# Autodesk Inventor assembly: Control Assembly Exploded
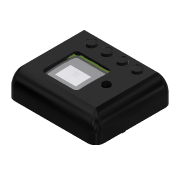
[picture p0: Inventor's stored thumbnail of the model, 180x180]
Saved by Autodesk Inventor 2017 (Build 210142000, 142)
## iProperties
Created: 2016-12-22
Part Number: Control Assembly Exploded
Document SubType Name: Assembly
Designer: ge937963
Author: ge937963
## Documents named in this file (15)
- C:\Users\ge937963\Desktop\Inventor View\Control Assembly.iam
- C:\Users\ge937963\Desktop\Inventor View\Control Board.ipt
- C:\Users\ge937963\Desktop\Inventor View\7 Pin female.iam
- C:\Users\ge937963\Desktop\Inventor View\7 Pin Male.iam
- C:\Users\ge937963\Desktop\Inventor View\Faceplate.ipt
- C:\Users\ge937963\Desktop\Inventor View\Button Piece.ipt
- C:\Users\ge937963\Desktop\Inventor View\Button.ipt
- C:\Users\ge937963\Desktop\Inventor View\2 Pin Female.iam
- C:\Users\ge937963\Desktop\Inventor View\2 Pin Male.iam
- C:\Users\ge937963\Desktop\Inventor View\Power switch.ipt
- C:\Users\ge937963\Desktop\Inventor View\Main PCB.ipt
- C:\Users\ge937963\Desktop\Inventor View\8 Pin female.iam
- C:\Users\ge937963\Desktop\Inventor View\4 Pin Female.iam
- C:\Users\ge937963\Desktop\Inventor View\MicroView.ipt
- C:\Users\ge937963\Desktop\Inventor View\Screw.ipt
## Components (27 placed, 14 different names)
1. Control Board:1 — Mate:52, Mate:53
2. 7 Pin female:1 [sub-assembly] — Mate:48, Mate:49, Mate:51
3. 7 Pin Male:1 [sub-assembly] — Mate:48, Mate:49, Mate:51
4. Faceplate:1 — Mate:53
5. Button Piece:1
6. Button Piece:2
7. Button Piece:3
8. Button Piece:4
9. Button:1
10. Button:2
11. Button:3
12. Button:4
13. 2 Pin Female:1 [sub-assembly]
14. 2 Pin Male:1 [sub-assembly]
15. Power switch:1
16. Main PCB:1
17. 8 Pin female:1 [sub-assembly]
18. 8 Pin female:2 [sub-assembly] — Mate:50
19. 2 Pin Female:2 [sub-assembly]
20. 4 Pin Female:1 [sub-assembly]
21. 4 Pin Female:2 [sub-assembly]
22. 2 Pin Female:3 [sub-assembly]
23. 2 Pin Female:4 [sub-assembly]
24. MicroView:1 — Mate:50
25. Screw:1 — Mate:52
26. Screw:2
27. Screw:3
## Relationships (71: Mate 53, Flush 16, Angle 2)
- [Mate]: Control Board:1 ↔ 7 Pin Male:1
- [Mate]: Control Board:1 ↔ 7 Pin Male:1
- [Mate]: Control Board:1 ↔ Faceplate:1
- [Mate]: Control Board:1 ↔ Faceplate:1
- [Flush]: Button Piece:1 ↔ Button Piece:2
- [Flush]: Button Piece:2 ↔ Button Piece:3
- [Flush]: Button Piece:3 ↔ Button Piece:4
- [Mate]: Faceplate:1 ↔ Button Piece:1
- [Mate]: Faceplate:1 ↔ Button Piece:2
- [Mate]: Faceplate:1 ↔ Button Piece:3
- [Mate]: Faceplate:1 ↔ Button Piece:4
- [Mate]: Control Board:1 ↔ 7 Pin Male:1
- [Flush]: Button:1 ↔ Button:2
- [Flush]: Button:2 ↔ Button:3
- [Flush]: Button:3 ↔ Button:4
- [Mate]: Control Board:1 ↔ Button:3
- [Mate]: Button Piece:4 ↔ Button:1
- [Mate]: Button Piece:3 ↔ Button:2
- [Flush]: Button:3 ↔ Button:4
- [Flush]: Button:2 ↔ Button:3
- [Flush]: Button:1 ↔ Button:2
- [Mate]: Control Board:1 ↔ 2 Pin Female:1
- [Mate]: Control Board:1 ↔ 2 Pin Female:1
- [Mate]: Control Board:1 ↔ 2 Pin Male:1
- [Mate]: Control Board:1 ↔ 2 Pin Male:1
- [Mate]: Control Board:1 ↔ 2 Pin Male:1
- [Mate]: Control Board:1 ↔ 2 Pin Female:1
- [Mate]: Control Board:1 ↔ Power switch:1
- [Mate]: Faceplate:1 ↔ Power switch:1
- [Angle] (0 deg): Control Board:1 ↔ Power switch:1
- [Mate]: Button Piece:2 ↔ Button:3
- [Mate]: Button Piece:1 ↔ Button:4
- [Mate]: 7 Pin female:1 ↔ Main PCB:1
- [Mate]: 7 Pin female:1 ↔ Main PCB:1
- [Mate]: 7 Pin female:1 ↔ Main PCB:1
- [Mate]: Main PCB:1 ↔ 8 Pin female:1
- [Mate]: Main PCB:1 ↔ 8 Pin female:2
- [Mate]: Main PCB:1 ↔ 8 Pin female:2
- [Mate]: Main PCB:1 ↔ 8 Pin female:1
- [Mate]: Main PCB:1 ↔ 8 Pin female:1
- [Flush]: 8 Pin female:1 ↔ 8 Pin female:2
- [Mate]: Main PCB:1 ↔ 2 Pin Female:2
- [Mate]: Main PCB:1 ↔ 2 Pin Female:2
- [Mate]: Main PCB:1 ↔ 2 Pin Female:2
- [Mate]: Main PCB:1 ↔ 4 Pin Female:1
- [Mate]: Main PCB:1 ↔ 4 Pin Female:1
- [Mate]: Main PCB:1 ↔ 4 Pin Female:2
- [Mate]: Main PCB:1 ↔ 4 Pin Female:2
- [Mate]: Main PCB:1 ↔ 4 Pin Female:2
- [Mate]: Main PCB:1 ↔ 4 Pin Female:1
- [Mate]: Main PCB:1 ↔ 2 Pin Female:3
- [Mate]: Main PCB:1 ↔ 2 Pin Female:3
- [Mate]: Main PCB:1 ↔ 2 Pin Female:4
- [Mate]: Main PCB:1 ↔ 2 Pin Female:4
- [Flush]: 4 Pin Female:2 ↔ 2 Pin Female:4
- [Flush]: 4 Pin Female:2 ↔ 2 Pin Female:3
- [Angle] (0 deg): 8 Pin female:2 ↔ MicroView:1
- [Flush] (-1.016 mm): 8 Pin female:1 ↔ MicroView:1
- [Flush] (-1.016 mm): 8 Pin female:1 ↔ MicroView:1
- [Mate]: Button Piece:4 ↔ Button:1
- [Mate]: Control Board:1 ↔ Screw:1
- [Mate]: Control Board:1 ↔ Screw:3
- [Mate]: Control Board:1 ↔ Screw:2
- [Flush]: Screw:2 ↔ Screw:3
- [Flush]: Screw:1 ↔ Screw:3
- Mate:48: 7 Pin female:1 ↔ 7 Pin Male:1
- Mate:49: 7 Pin female:1 ↔ 7 Pin Male:1
- Mate:50: 8 Pin female:2 ↔ MicroView:1
- Mate:51: 7 Pin female:1 ↔ 7 Pin Male:1
- Mate:52: Control Board:1 ↔ Screw:1
- Mate:53: Control Board:1 ↔ Faceplate:1
## Named parameters: d32_d61 = 0 mm, d33_d63 = 0 mm, d34_d64 = 0 mm
